# Autodesk Inventor assembly: Build Platform Assembly - Double Z - 1.0
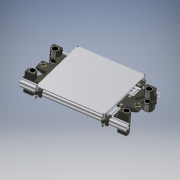
[picture p0: Inventor's stored thumbnail of the model, 180x180]
Saved by Autodesk Inventor 2016 (Build 200138000, 138)
## iProperties
Created: 2017-04-14
Part Number: Build Platform Assembly - Double Z - 1.0
Document SubType Name: Assembly
Designer: Scott
Author: Scott
## Documents named in this file (8)
- E:\Scott Projects\3D Printing\CoreXY\Build Platform Assembly - Double Z - 1.0.iam
- E:\Scott Projects\3D Printing\CoreXY\2020 Extrusion - Double Z motor - Bed X.ipt
- E:\Scott Projects\3D Printing\CoreXY\2020 Extrusion - Double Z motor - Bed Y.ipt
- E:\Scott Projects\3D Printing\CoreXY\Z Axis Bearing Holder 1.0.ipt
- E:\Scott Projects\3D Printing\CoreXY\LM12UU.ipt
- E:\Scott Projects\3D Printing\CoreXY\Heated Bed.ipt
- E:\Scott Projects\3D Printing\CoreXY\Z Nut Bracket Assemby 1.0.iam
- E:\Scott Projects\3D Printing\CoreXY\Bed Bracket 1.0.iam
## Components (23 placed, 7 different names)
1. 2020 Extrusion - Double Z motor - Bed X:1 — Mate:3, Flush:2, Flush:4, Mate:5, Flush:5, Mate:7, Mate:8, Flush:6, Mate:12, Flush:9, Mate:15, Flush:14, Mate:27, Mate:28, Mate:29, Mate:31
2. 2020 Extrusion - Double Z motor - Bed X:2 — Mate:4, Flush:3, Flush:4, Mate:10, Flush:7, Mate:14, Flush:11, Mate:21, Mate:22, Mate:24, Mate:25
3. 2020 Extrusion - Double Z motor - Bed Y:1 — Mate:3, Flush:2, Mate:4, Flush:3, Mate:11, Mate:13, Flush:13, Mate:16, Mate:17, Mate:18
4. 2020 Extrusion - Double Z motor - Bed Y:2 — Mate:5, Flush:5, Mate:6, Mate:9, Mate:19, Mate:20, Flush:15
5. Z Axis Bearing Holder 1.0:1 — Mate:11, Mate:12, Flush:9, Flush:10, Insert:4, Insert:5
6. Z Axis Bearing Holder 1.0:2 — Mate:13, Mate:14, Flush:11, Flush:12, Insert:3, Insert:6
7. Z Axis Bearing Holder 1.0:3 — Mate:9, Mate:10, Flush:7, Flush:8, Insert:2, Insert:7
8. Z Axis Bearing Holder 1.0:4 — Mate:6, Mate:7, Mate:8, Flush:6, Flush:8, Flush:10, Flush:12, Insert:1, Insert:8
9. LM12UU:1 — Insert:1
10. LM12UU:2 — Insert:2
11. LM12UU:3 — Insert:4
12. LM12UU:4 — Insert:3
13. LM12UU:5 — Insert:6
14. LM12UU:6 — Insert:5
15. LM12UU:7 — Insert:7
16. LM12UU:8 — Insert:8
17. Heated Bed:1 — Mate:15, Flush:13, Flush:14, Mate:23, Mate:26, Mate:30, Mate:32
18. Z Nut Bracket Assemby 1.0:1 [sub-assembly] — Mate:16, Mate:17, Mate:18
19. Z Nut Bracket Assemby 1.0:2 [sub-assembly] — Mate:19, Mate:20, Flush:15
20. Bed Bracket 1.0:1 [sub-assembly] — Mate:21, Mate:22, Mate:23
21. Bed Bracket 1.0:2 [sub-assembly] — Mate:24, Mate:25, Mate:26
22. Bed Bracket 1.0:3 [sub-assembly] — Mate:28, Mate:29, Mate:30
23. Bed Bracket 1.0:4 [sub-assembly] — Mate:27, Mate:31, Mate:32
## Relationships (52: Mate 30, Flush 14, Insert 8)
- Mate:3: 2020 Extrusion - Double Z motor - Bed X:1 ↔ 2020 Extrusion - Double Z motor - Bed Y:1
- Flush:2: 2020 Extrusion - Double Z motor - Bed X:1 ↔ 2020 Extrusion - Double Z motor - Bed Y:1
- Mate:4: 2020 Extrusion - Double Z motor - Bed X:2 ↔ 2020 Extrusion - Double Z motor - Bed Y:1
- Flush:3: 2020 Extrusion - Double Z motor - Bed X:2 ↔ 2020 Extrusion - Double Z motor - Bed Y:1
- Flush:4: 2020 Extrusion - Double Z motor - Bed X:1 ↔ 2020 Extrusion - Double Z motor - Bed X:2
- Mate:5: 2020 Extrusion - Double Z motor - Bed X:1 ↔ 2020 Extrusion - Double Z motor - Bed Y:2
- Flush:5: 2020 Extrusion - Double Z motor - Bed X:1 ↔ 2020 Extrusion - Double Z motor - Bed Y:2
- Mate:6: 2020 Extrusion - Double Z motor - Bed Y:2 ↔ Z Axis Bearing Holder 1.0:4
- Mate:7: 2020 Extrusion - Double Z motor - Bed X:1 ↔ Z Axis Bearing Holder 1.0:4
- Mate:8 (0.2 mm): 2020 Extrusion - Double Z motor - Bed X:1 ↔ Z Axis Bearing Holder 1.0:4
- Flush:6: 2020 Extrusion - Double Z motor - Bed X:1 ↔ Z Axis Bearing Holder 1.0:4
- Mate:9: 2020 Extrusion - Double Z motor - Bed Y:2 ↔ Z Axis Bearing Holder 1.0:3
- Mate:10: 2020 Extrusion - Double Z motor - Bed X:2 ↔ Z Axis Bearing Holder 1.0:3
- Flush:7: 2020 Extrusion - Double Z motor - Bed X:2 ↔ Z Axis Bearing Holder 1.0:3
- Flush:8: Z Axis Bearing Holder 1.0:3 ↔ Z Axis Bearing Holder 1.0:4
- Mate:11: 2020 Extrusion - Double Z motor - Bed Y:1 ↔ Z Axis Bearing Holder 1.0:1
- Mate:12: 2020 Extrusion - Double Z motor - Bed X:1 ↔ Z Axis Bearing Holder 1.0:1
- Flush:9: 2020 Extrusion - Double Z motor - Bed X:1 ↔ Z Axis Bearing Holder 1.0:1
- Flush:10: Z Axis Bearing Holder 1.0:1 ↔ Z Axis Bearing Holder 1.0:4
- Mate:13: 2020 Extrusion - Double Z motor - Bed Y:1 ↔ Z Axis Bearing Holder 1.0:2
- Mate:14: 2020 Extrusion - Double Z motor - Bed X:2 ↔ Z Axis Bearing Holder 1.0:2
- Flush:11: 2020 Extrusion - Double Z motor - Bed X:2 ↔ Z Axis Bearing Holder 1.0:2
- Flush:12: Z Axis Bearing Holder 1.0:2 ↔ Z Axis Bearing Holder 1.0:4
- Insert:1: Z Axis Bearing Holder 1.0:4 ↔ LM12UU:1
- Insert:2: Z Axis Bearing Holder 1.0:3 ↔ LM12UU:2
- Insert:3: Z Axis Bearing Holder 1.0:2 ↔ LM12UU:4
- Insert:4: Z Axis Bearing Holder 1.0:1 ↔ LM12UU:3
- Insert:5: Z Axis Bearing Holder 1.0:1 ↔ LM12UU:6
- Insert:6: Z Axis Bearing Holder 1.0:2 ↔ LM12UU:5
- Insert:7: Z Axis Bearing Holder 1.0:3 ↔ LM12UU:7
- Insert:8: Z Axis Bearing Holder 1.0:4 ↔ LM12UU:8
- Mate:15 (20 mm): 2020 Extrusion - Double Z motor - Bed X:1 ↔ Heated Bed:1
- Flush:13: 2020 Extrusion - Double Z motor - Bed Y:1 ↔ Heated Bed:1
- Flush:14: 2020 Extrusion - Double Z motor - Bed X:1 ↔ Heated Bed:1
- Mate:16: 2020 Extrusion - Double Z motor - Bed Y:1 ↔ Z Nut Bracket Assemby 1.0:1
- Mate:17: 2020 Extrusion - Double Z motor - Bed Y:1 ↔ Z Nut Bracket Assemby 1.0:1
- Mate:18: 2020 Extrusion - Double Z motor - Bed Y:1 ↔ Z Nut Bracket Assemby 1.0:1
- Mate:19: 2020 Extrusion - Double Z motor - Bed Y:2 ↔ Z Nut Bracket Assemby 1.0:2
- Mate:20: 2020 Extrusion - Double Z motor - Bed Y:2 ↔ Z Nut Bracket Assemby 1.0:2
- Flush:15: 2020 Extrusion - Double Z motor - Bed Y:2 ↔ Z Nut Bracket Assemby 1.0:2
- Mate:21: 2020 Extrusion - Double Z motor - Bed X:2 ↔ Bed Bracket 1.0:1
- Mate:22: 2020 Extrusion - Double Z motor - Bed X:2 ↔ Bed Bracket 1.0:1
- Mate:23: Heated Bed:1 ↔ Bed Bracket 1.0:1
- Mate:24: 2020 Extrusion - Double Z motor - Bed X:2 ↔ Bed Bracket 1.0:2
- Mate:25: 2020 Extrusion - Double Z motor - Bed X:2 ↔ Bed Bracket 1.0:2
- Mate:26: Heated Bed:1 ↔ Bed Bracket 1.0:2
- Mate:27: 2020 Extrusion - Double Z motor - Bed X:1 ↔ Bed Bracket 1.0:4
- Mate:28: 2020 Extrusion - Double Z motor - Bed X:1 ↔ Bed Bracket 1.0:3
- Mate:29: 2020 Extrusion - Double Z motor - Bed X:1 ↔ Bed Bracket 1.0:3
- Mate:30: Heated Bed:1 ↔ Bed Bracket 1.0:3
- Mate:31: 2020 Extrusion - Double Z motor - Bed X:1 ↔ Bed Bracket 1.0:4
- Mate:32: Heated Bed:1 ↔ Bed Bracket 1.0:4
